# Autodesk Inventor assembly: Curved Assembly
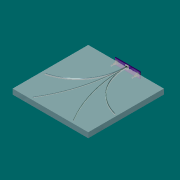
[picture p0: Inventor's stored thumbnail of the model, 180x180]
Saved by Autodesk Inventor 2016 (Build 200138000, 138)
## iProperties
Created: 2015-08-14
Part Number: Curved Assembly
Document SubType Name: Assembly
Designer: Cosmic
Author: Cosmic
## Documents named in this file (8)
- C:\Users\Sawaiz\Documents\data\projects\scintillatorPanel\treePanel.iam
- C:\Users\Sawaiz\Documents\data\projects\scintillatorPanel\treePanel.ipt
- C:\Users\Sawaiz\Documents\data\projects\scintillatorPanel\treeFiberBundle.iam
- C:\Users\Sawaiz\Documents\data\projects\scintillatorPanel\mppcSensorInterface\cad\sensor.iam
- C:\Users\Sawaiz\Documents\data\projects\scintillatorPanel\m3x8.ipt
- C:\Users\Sawaiz\Documents\data\projects\scintillatorPanel\2mmSpacer.ipt
- C:\Users\Sawaiz\Documents\data\projects\scintillatorPanel\m3Washer.ipt
- C:\Users\Sawaiz\Documents\data\projects\scintillatorPanel\Scintillator.xlsx
## Components (9 placed, 6 different names)
1. treePanel:1 — Angle:1, Tangent:2, Flush:1, Mate:14, Mate:20, Mate:22, Mate:27
2. treeFiberBundle:1 [sub-assembly] — Angle:1, Tangent:2, Flush:1, Mate:27
3. sensor:1 [sub-assembly] — Mate:12, Mate:15, Mate:17, Mate:18, Mate:24, Mate:25
4. m3x8:1 — Mate:17, Mate:24, Mate:26
5. m3x8:2 — Mate:18, Mate:19, Mate:21, Mate:25
6. 2mmSpacer:1 — Mate:16, Mate:22, Mate:23, Mate:26
7. 2mmSpacer:2 — Mate:13, Mate:14, Mate:19
8. m3Washer:1 — Mate:15, Mate:16, Mate:23
9. m3Washer:2 — Mate:12, Mate:13, Mate:20, Mate:21
## Relationships (19: Mate 16, Angle 1, Tangent 1, Flush 1)
- Angle:1 (-90 deg): treePanel:1 ↔ treeFiberBundle:1
- Tangent:2 (0.15 mm): treePanel:1 ↔ treeFiberBundle:1
- Flush:1: treePanel:1 ↔ treeFiberBundle:1
- Mate:12: sensor:1 ↔ m3Washer:2
- Mate:13: 2mmSpacer:2 ↔ m3Washer:2
- Mate:14: treePanel:1 ↔ 2mmSpacer:2
- Mate:15: sensor:1 ↔ m3Washer:1
- Mate:16: 2mmSpacer:1 ↔ m3Washer:1
- Mate:17: sensor:1 ↔ m3x8:1
- Mate:18: sensor:1 ↔ m3x8:2
- Mate:19: m3x8:2 ↔ 2mmSpacer:2
- Mate:20: treePanel:1 ↔ m3Washer:2
- Mate:21: m3x8:2 ↔ m3Washer:2
- Mate:22: treePanel:1 ↔ 2mmSpacer:1
- Mate:23: 2mmSpacer:1 ↔ m3Washer:1
- Mate:24: sensor:1 ↔ m3x8:1
- Mate:25: sensor:1 ↔ m3x8:2
- Mate:26: m3x8:1 ↔ 2mmSpacer:1
- Mate:27: treePanel:1 ↔ treeFiberBundle:1
## Named parameters: OpticalFiberClearence = 0.15 mm, MPPCClearence = 0.075 mm, FiberSensorClerence = 0.5 mm, OpticalFiberDiameter = 1 mm, ScintillatorThickness = 10 mm, SmallTrackDiameter = 175 mm, LargeTrackRatio = 3, ScintillatorEdgeClearence = 3 mm, ScintillatorWidth = 145 mm, ScintillatorHeight = 145 mm, ShallowTrackDepth = 1.3 mm, MPPCSensorClearence = 1.45 mm, MPPCSensorOffsett = 2.105 mm, MPPCWidth = 5.9 mm, MPPCHeight = 6.55 mm, FiberEdgeOffsett = 5 mm, MPPCDepth = 0 mm, LongFiberAngle = 30 deg, ShortFiberAngle = 78 deg, LoopLargeTrackRatio = 1.1, LoopSmallTrackDiameter = 90 mm, MountingScrewOffsett = 20 mm, MountingScrewDepth = 4 mm
